# Autodesk Inventor assembly: Display_CCM_Mount
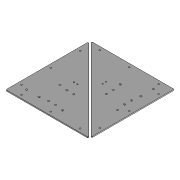
[picture p0: Inventor's stored thumbnail of the model, 180x180]
Saved by Autodesk Inventor 2020 (Build 240168000, 168)
## iProperties
Created: 2021-07-28
Part Number: Display_CCM_Mount
Document SubType Name: Assembly
Designer: magnarecta
Author: magnarecta
## Documents named in this file (2)
- C:\Users\lvglv\Documents\GitHub\Eto_Project\Hardware\Parts\Meviy\Meviy_Asem\Display_CCM_Mount.iam
- C:\Users\lvglv\Documents\GitHub\Eto_Project\Hardware\Parts\Meviy\Display_CCM_Mount.ipt
## Components (2 placed, 1 different names)
1. Display_CCM_Mount:1 — メイト:1, フラッシュ:1
2. Display_CCM_Mount:2 — メイト:1, フラッシュ:1
## Relationships (2: Mate 1, Flush 1)
- メイト:1 [Mate] (5 mm): Display_CCM_Mount:1 ↔ Display_CCM_Mount:2
- フラッシュ:1 [Flush]: Display_CCM_Mount:1 ↔ Display_CCM_Mount:2
